# Autodesk Inventor assembly: 042-DXDE(F,D-166-3)
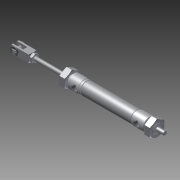
[picture p0: Inventor's stored thumbnail of the model, 180x180]
Saved by Autodesk Inventor 2012 (Build 160160000, 160)
## iProperties
Created: 2013-01-17
Part Number: 042-DXDE(F,D-166-3)
Catalog Web Link: www.cadenas.de
Description: Original Line Standard Air Cylinders-
Vendor: BIMBA
Document SubType Name: Assembly
Designer: William
Manufacturer: BIMBA
Category: PARTsolutions
Company: BIMBA
Title: 042-DXDE
Author: Cadenas PARTsolutions
PSOL_IDENT_0: {\\10.0.0.242\data_v9\23d-libs\bimba\bimba\bimba_imperial\bimba_full_line\original_line_cylinders\st
PSOL_IDENT_1: andard_air_cylinders\standard_air_cylinder_asmtab.prj},318 {VTYP=3D},{STYP=ASSTAB},{NB=042-DXDE(F,D-
PSOL_IDENT_2: 166-3)},{LINA=042-DXDE},{NN=Original Line Standard Air Cylinders},{DATE=06.09.2012 11:26:56},{GEOMDA
PSOL_IDENT_3: TE=06.09.2012},{VERSION=},{LINEID=50},{LINESUBID=-1},{WBVAR=STROKE,ACTING,MNT,DER,NR,BM,CO,OO,VO,M,E
PSOL_IDENT_4: E,EEL,K,Q,Y,G,T,B,H,SER,SR,NT,W,HL,STPT1,STPT2,STPT3,STPT4,MB,PB,PRC,TB,MN}  {NB=042-DXDE(F,D-166-3)
PSOL_IDENT_5: },{LINA=042-DXDE},{KT=DUMMY},{PN=042-DXDE},{PNC=042-DXDE(F,D-166-3)},{PNA=(D-166-3)},{DASH=-},{BORE1
PSOL_IDENT_6: =0.75000000},{BORE=3/4\" (04)},{BOREPN=04},{STROKE=2.000},{STROKEALG=[0.011:50/0.001]},{STROKE1=2.00
PSOL_IDENT_7: 0},{ACTING=D},{ACTINGALG= '' , 'Single Acting (SA)' , 'R' , 'Reverse Single Acting (SA)' , 'D' , 'Do
PSOL_IDENT_8: uble Acting (SA)' },{ACTINGPN=D},{MNT=X},{MNTALG= '' , 'Front Nose Mounting (SA)' , 'P' , 'Rear Pivo
PSOL_IDENT_9: t Mounting (SA)' , 'XP' , 'Double End or Pivot Mounting (SA)' , 'X' , 'Double End Mounting (SA)' , '
PSOL_IDENT_10: BF' , 'Front Block Mounting (SA)' , 'BR' , 'Rear Block Mounting for Vertical Positioning (SA)' , 'BF
PSOL_IDENT_11: T' , 'Front Block Trunnion Mounting (SA)' , 'BRT' , 'Rear Block Trunnion Mounting (SA)' },{TYPE=},{M
PSOL_IDENT_12: NTPN=X},{DER=DE},{DERALG= 'DE' , 'With Double End Rod' },{NR=},{NRALG= '' , 'N/A' },{NRPN=},{BM=},{B
PSOL_IDENT_13: MALG= '' , 'N/A' },{BMPN=},{CO=},{COALG= '' , 'N/A' },{OO=},{OOALG= '', 'N/A' },{OOPN=},{VO=Z},{VOAL
PSOL_IDENT_14: G= 'Z' , 'N/A' },{VOPN=},{OOVOPN=},{M=},{MALG= '', 'Without Magnet', 'M', 'With Magnet' },{EE=},{EEL
PSOL_IDENT_15: =0.000},{EEMAX=48.0000},{EEALG= '', 'Without Extra Extension', 'EE', 'With Extra Extension' },{EELAL
PSOL_IDENT_16: G=0},{EEPN=},{EEPN1=0.000},{K=},{KALG= '' , 'N/A' },{KPN=},{Q=},{QALG= '' , 'N/A' },{QPN=},{Y=},{YAL
PSOL_IDENT_17: G= '' , 'N/A' },{YPN=},{YCON=},{F=},{FALG= '', 'Non-Coated (Standard)', 'F', 'Molycoated' },{FPN=},{
PSOL_IDENT_18: G=},{GPN=},{GPN99=},{T=},{TALG= '' , 'Standard -20° to 200°F (-29° to 95°C)' , 'N' , 'Low Temperatur
PSOL_IDENT_19: e' , 'V' , 'High Temperature' },{NPN=},{VPN=},{B=},{BALG= '', 'W/out Bumpers' , 'B' , 'W/ Bumpers' }
PSOL_IDENT_20: ,{BPN=},{H=},{HALG= '', 'N/A' },{HPN=},{SER=},{SERALG= '' , 'Without Spring Return' , 'JS' , 'With S
PSOL_IDENT_21: pring Return' },{SR=},{SRALG= '' , 'Standard Stainless Steel' },{SRPN=},{SRCON=0},{NT=},{NTPN=},{W=}
PSOL_IDENT_22: ,{WALG= '' , 'Without Wiper' , 'W' , 'With Wiper' },{WPN=},{E=},{EALG= '' , 'Standard Seals/Lube' ,
PSOL_IDENT_23: 'E' , 'Non-Lube Seals/Lube' },{EPN=},{HL=},{HLALG= '' , 'Without Low Pressure Hydraulic' , 'HL' , 'W
PSOL_IDENT_24: ith Low Pressure Hydraulic' },{ST=},{STALG= '' , 'N/A' },{STPT1=},{STPT1ALG= '' , 'N/A' },{STPT2=},{
PSOL_IDENT_25: STPT2ALG= '' , 'N/A' },{STPT3=},{STPT3ALG= '' , 'N/A' },{STPT4=},{STPT4ALG= '' , 'N/A' },{STPN=},{MB
PSOL_IDENT_26: =},{MBALG= '' , 'Without Mounting Bracket' , 'F,D-129' , 'D-129 (front)'  , 'R,D-129' , 'D-129 (rear
PSOL_IDENT_27: )' , '2x,D-129' , 'D-129 (front & rear)'},{MBPN=},{MBPNALL=D-129},{MBPNALLREAR=D-129},{PB=},{PBALG=
PSOL_IDENT_28: '' , 'N/A' },{PBPN=},{PBPNALL=},{PRC=F,D-166-3},{PRCALG= '' , 'W/out Pivot Rod Clevis' , 'F,D-166-3'
PSOL_IDENT_29: , 'D-166-3 (front)' , 'R,D-166-3' , 'D-166-3 (rear)' , '2x,D-166-3' , 'D-166-3 (front & rear)' },{P
PSOL_IDENT_30: RCPN=(F,D-166-3)},{PRCPNALL=D-166-3},{TB=},{TBALG= '' , 'N/A' },{TBPN=},{TBPNALL=},{MN=},{MNALG= ''
PSOL_IDENT_31: , 'N/A' },{MNPN=},{MNCONF=},{MNCONR=},{TLEN=3.2570},{FRAC=9.0000},{RGCON=},{RGDACCON=R},{RHCON=DX},{
PSOL_IDENT_32: RHCON1=DX},{RHCONON=0},{RHACCON=},{FNUTCON=1},{RNUTCON=1},{FNUTPN=D-9},{RNUTPN=D-9},{FNUTTRANS=0.000
PSOL_IDENT_33: 0},{RNUTTRANS=0.0000},{VHOLECON=0},{A1=1.5940},{A1N=0.8750},{A1P=1.5940},{A1B=1.5940},{A4=0.2525},{A
PSOL_IDENT_34: 4N=0.3130},{A4P=0.2525},{A5=0.0300},{A1H=1.594},{A1NH=0.5310},{A1PH=1.5940},{A1BH=1.0940},{A1SH=1.21
PSOL_IDENT_35: 90},{A2H=0.2190},{A2NH=0.2190},{LENGTH=4.0000},{LENGTH1=4.0000},{LENGTH2=0.0000},{MUL=2.0000},{MUL11
PSOL_IDENT_36: =2.0000},{MUL22=5.38},{MUL33=5.3800},{MUL2=2.0000},{MUL211=2.0000},{MUL222=2.6900},{MUL233=2.6900},{
PSOL_IDENT_37: SSS=4.0000},{RGLEN=1.3715},{RHLEN=1.3715},{SSS1=3.0000},{A13=1.3120},{DIF=0.0000},{G5=0.6250},{ON=0}
PSOL_IDENT_38: ,{SSADD=0.0000},{BADD=0.0000},{MADD=0.0000},{NVADD=0.0000},{TRACKL=2.9670},{TRACKCON=D-74168},{TRIMC
PSOL_IDENT_39: ON=0},{TRIMCON1=0},{PINCON=},{FSPACE=0.6926},{SPACE=0.0643},{TEXT=0.1125},{S1=1.0000},{D1=0.8325},{D
PSOL_IDENT_40: 1N=0.8050},{D1B=0.8625},{D1P=0.8325},{FA=0.940},{RA=0.9400},{PPATH=standard_air_cylinder_asmtpl.prj}
PSOL_IDENT_41: ,{MATALGHTML=<b>Standard Original Line:</b><dl><dt>Rod:</dt><dd>- Stainless Steel</dd><dd>&nbsp;&nbs
PSOL_IDENT_42: p;(5/16  9/16 Bores)</dd><dd>- High Strength Carbon Steel</dd><dd>&nbsp;&nbsp;(3/4  3 Bore)</dd><d
PSOL_IDENT_43: d>- Stainless Steel</dd><dd>&nbsp;&nbsp;(X style DXP/DX/DXDE)</dd><dt>Bearings:</dt><dd>- Sintere
PSOL_IDENT_44: d Bronze</dd><dt>Body:</dt><dd>- 304 Stainless Steel</dd><dt>End Caps:</dt><dd>- Aluminum</dd><dt>Se
PSOL_IDENT_45: als:</dt><dd>- Buna N</dd></dl>},{ASSCFGPRA=04DXDE},{MBPNA=},{MNPNA=},{PRCPNA=(D-166-3)},{ASSOPTACC=
PSOL_IDENT_46: STPT4},{A=8.00},{HADD=0.0000},{WFL=0.25},{QADD=0.000},{QADD1=0.440},{TEST=2.0000},{MNTB=},{STDNUTF=1
PSOL_IDENT_47: },{STDNUTR=1}
CNS_NT: Standard Male Thread
CNS_NB: 042-DXDE(F,D-166-3)
CNS_NBSYN: $PNC.
CNS_LINA: 042-DXDE
CNS_PN: 042-DXDE
CNS_PNC: 042-DXDE(F,D-166-3)
CNS_PNA: (D-166-3)
CNS_DASH: -
CNS_BORE1: 0.75000000
CNS_BORE: 3/4" [04]
CNS_BOREPN: 04
CNS_STROKE: 2.000
CNS_STROKEALG: [0.011:50/0.001]
CNS_STROKE1: 2.000
CNS_ACTING: Double [D]
CNS_ACTINGALG: '' , 'Single Acting (SA)' , 'R' , 'Reverse Single Acting (SA)' , 'D' , 'Double Acting (SA)'
CNS_ACTINGPN: D
CNS_MNT: Double End [X]
CNS_MNTALG: '' , 'Front Nose Mounting (SA)' , 'P' , 'Rear Pivot Mounting (SA)' , 'XP' , 'Double End or Pivot Mounting (SA)' , 'X' , 'Double End Mounting (SA)' , 'BF' , 'Front Block Mounting (SA)' , 'BR' , 'Rear Block Mounting for Vertical Positioning (SA)' , 'BFT' , 'Front Block Trunnion Mounting (SA)' , 'BRT' , 'Rear Block Trunnion Mounting (SA)'
CNS_MNTPN: X
CNS_DER: Double End Rod [DE]
CNS_DERALG: 'DE' , 'With Double End Rod'
CNS_NR: N/A
CNS_NRALG: '' , 'N/A'
CNS_BM: N/A
CNS_BMALG: '' , 'N/A'
CNS_CO: N/A
CNS_COALG: '' , 'N/A'
CNS_OO: N/A
CNS_OOALG: '', 'N/A'
CNS_VO: N/A
CNS_VOALG: 'Z' , 'N/A'
CNS_M: Without Magnet Piston
CNS_MALG: '', 'Without Magnet', 'M', 'With Magnet'
CNS_EE: Standard Rod Extension
CNS_EEL: 0.000
CNS_EEMAX: 48.0000
CNS_EEALG: '', 'Without Extra Extension', 'EE', 'With Extra Extension'
CNS_EELALG: 0
CNS_EEPN1: 0.000
CNS_K: N/A
CNS_KALG: '' , 'N/A'
CNS_Q: N/A
CNS_QALG: '' , 'N/A'
CNS_Y: N/A
CNS_YALG: '' , 'N/A'
CNS_FALG: '', 'Non-Coated (Standard)', 'F', 'Molycoated'
CNS_G: Standard Grease Lube
CNS_T: Standard -20° to 200°F (-29° to 95°C)
CNS_TALG: '' , 'Standard -20° to 200°F (-29° to 95°C)' , 'N' , 'Low Temperature' , 'V' , 'High Temperature'
CNS_B: Without Bumpers
CNS_BALG: '', 'W/out Bumpers' , 'B' , 'W/ Bumpers'
CNS_H: N/A
CNS_HALG: '', 'N/A'
CNS_SER: Without Failsafe Spring Return
CNS_SERALG: '' , 'Without Spring Return' , 'JS' , 'With Spring Return'
CNS_SR: Standard Stainless Steel
CNS_SRALG: '' , 'Standard Stainless Steel'
CNS_SRCON: 0
CNS_W: Without Wiper
CNS_WALG: '' , 'Without Wiper' , 'W' , 'With Wiper'
CNS_EALG: '' , 'Standard Seals/Lube' , 'E' , 'Non-Lube Seals/Lube'
CNS_HL: Standard 250 PSI Air
CNS_HLALG: '' , 'Without Low Pressure Hydraulic' , 'HL' , 'With Low Pressure Hydraulic'
CNS_STALG: '' , 'N/A'
CNS_STPT1: N/A
CNS_STPT1ALG: '' , 'N/A'
CNS_STPT2: N/A
CNS_STPT2ALG: '' , 'N/A'
CNS_STPT3: N/A
CNS_STPT3ALG: '' , 'N/A'
CNS_STPT4: N/A
CNS_STPT4ALG: '' , 'N/A'
CNS_MB: Without Mounting Bracket
CNS_MBALG: '' , 'Without Mounting Bracket' , 'F,D-129' , 'D-129 (front)'  , 'R,D-129' , 'D-129 (rear)' , '2x,D-129' , 'D-129 (front & rear)'
CNS_MBPNALL: D-129
CNS_MBPNALLREAR: D-129
CNS_PB: N/A
CNS_PBALG: '' , 'N/A'
CNS_PRC: D-166-3 (front)
CNS_PRCALG: '' , 'W/out Pivot Rod Clevis' , 'F,D-166-3' , 'D-166-3 (front)' , 'R,D-166-3' , 'D-166-3 (rear)' , '2x,D-166-3' , 'D-166-3 (front & rear)'
CNS_PRCPN: (F,D-166-3)
CNS_PRCPNALL: D-166-3
CNS_TB: N/A
CNS_TBALG: '' , 'N/A'
CNS_MN: N/A
CNS_MNALG: '' , 'N/A'
CNS_TLEN: 3.2570
CNS_FRAC: 9.0000
CNS_RGDACCON: R
CNS_RHCON: DX
CNS_RHCON1: DX
CNS_RHCONON: 0
CNS_FNUTCON: 1
CNS_RNUTCON: 1
CNS_FNUTPN: D-9
CNS_RNUTPN: D-9
CNS_FNUTTRANS: 0.0000
CNS_RNUTTRANS: 0.0000
CNS_VHOLECON: 0
CNS_A1: 1.5940
CNS_A1N: 0.8750
CNS_A1P: 1.5940
CNS_A1B: 1.5940
CNS_A4: 0.2525
CNS_A4N: 0.3130
CNS_A4P: 0.2525
CNS_A5: 0.0300
CNS_A1H: 1.594
CNS_A1NH: 0.5310
CNS_A1PH: 1.5940
CNS_A1BH: 1.0940
CNS_A1SH: 1.2190
CNS_A2H: 0.2190
CNS_A2NH: 0.2190
CNS_LENGTH: 4.0000
CNS_LENGTH1: 4.0000
CNS_LENGTH2: 0.0000
CNS_MUL: 2.0000
CNS_MUL11: 2.0000
CNS_MUL22: 5.380
CNS_MUL33: 5.3800
CNS_MUL2: 2.0000
CNS_MUL211: 2.0000
CNS_MUL222: 2.6900
CNS_MUL233: 2.6900
CNS_SSS: 4.0000
CNS_RGLEN: 1.3715
CNS_RHLEN: 1.3715
CNS_SSS1: 3.0000
CNS_A13: 1.3120
CNS_DIF: 0.0000
CNS_G5: 0.6250
CNS_ON: 0
CNS_SSADD: 0.0000
CNS_BADD: 0.0000
CNS_MADD: 0.0000
CNS_NVADD: 0.0000
CNS_TRACKL: 2.9670
CNS_TRACKCON: D-74168
CNS_TRIMCON: 0
CNS_TRIMCON1: 0
CNS_FSPACE: 0.6926
CNS_SPACE: 0.0643
CNS_TEXT: 0.1125
CNS_S1: 1.0000
CNS_D1: 0.8325
CNS_D1N: 0.8050
CNS_D1B: 0.8625
CNS_D1P: 0.8325
CNS_FA: 0.940
CNS_RA: 0.9400
CNS_PPATH: standard_air_cylinder_asmtpl.prj
CNS_MATALGHTML: <b>Standard Original Line:</b><dl><dt>Rod:</dt><dd>- Stainless Steel</dd><dd>&nbsp;&nbsp;(5/16  9/16 Bores)</dd><dd>- High Strength Carbon Steel</dd><dd>&nbsp;&nbsp;(3/4  3 Bore)</dd><dd>- Stainless Steel</dd><dd>&nbsp;&nbsp;(X style DXP/DX/DXDE)</dd><dt>Bearings:</dt><dd>- Sintered Bronze</dd><dt>Body:</dt><dd>- 304 Stainless Steel</dd><dt>End Caps:</dt><dd>- Aluminum</dd><dt>Seals:</dt><dd>- Buna N</dd></dl>
CNS_ASSCFGPRA: 04DXDE
CNS_PRCPNA: (D-166-3)
CNS_ASSOPTACC: STPT4
CNS_A: 8.00
CNS_HADD: 0.0000
CNS_WFL: 0.250
CNS_QADD: 0.000
CNS_QADD1: 0.440
CNS_TEST: 2.0000
CNS_STDNUTF: 1
CNS_STDNUTR: 1
SUPPLIER: BIMBA
ARTICLENO: 042-DXDE(F,D-166-3)
BOMINFO: 042-DXDE
CREATOR: CADENAS GmbH
## Documents named in this file (10)
- C:\Users\William\Desktop\FRC CAD Files\Robot2013\Launcher\042-DXDE(F,D-166-3).iam
- C:\Users\William\Desktop\FRC CAD Files\Robot2013\Launcher\04R000_rod_guide.ipt
- C:\Users\William\Desktop\FRC CAD Files\Robot2013\Launcher\042-DXDE0_rod.ipt
- C:\Users\William\Desktop\FRC CAD Files\Robot2013\Launcher\D-166-3-dummy.ipt
- C:\Users\William\Desktop\FRC CAD Files\Robot2013\Launcher\D-14055.ipt
- C:\Users\William\Desktop\FRC CAD Files\Robot2013\Launcher\D-8381.ipt
- C:\Users\William\Desktop\FRC CAD Files\Robot2013\Launcher\D-5866.ipt
- C:\Users\William\Desktop\FRC CAD Files\Robot2013\Launcher\D-344.ipt
- C:\Users\William\Desktop\FRC CAD Files\Robot2013\Launcher\04R-3_2570.ipt
- C:\Users\William\Desktop\FRC CAD Files\Robot2013\Launcher\D-9.ipt
## Components (12 placed, 9 different names)
1. 04R000_rod_guide:1 — rod_guide_Z@1 <-> rod_cp_Z@2, to_tube_XY@1 <-> tube_front_XY@9, to_tube_Z@1 <-> tube_front_Z@9, to_tube_YZ@1 <-> tube_front_YZ@9, to_nut_XY@1 <-> NUT_XY@12, to_nut_Z@1 <-> NUT_Z@12, to_nut_YZ@1 <-> NUT_YZ@12
2. 042-DXDE0_rod:1 — rod_guide_Z@1 <-> rod_cp_Z@2
3. D-166-3-dummy:1 — dummy_XY@3 <-> dummy_XY@4, dummy_Z@3 <-> dummy_Z@4, dummy_YZ@3 <-> dummy_YZ@4
4. D-14055:1 — dummy_XY@3 <-> dummy_XY@4, dummy_Z@3 <-> dummy_Z@4, dummy_YZ@3 <-> dummy_YZ@4, rod_clevis_body_XY@4 <-> pin_XY@5, rod_clevis_body_Z@4 <-> pin_Z@5, piston_rod_clevis_XY@4 <-> NUT_XY@8, piston_rod_clevis_Z@4 <-> NUT_Z@8
5. D-8381:1 — rod_clevis_body_XY@4 <-> pin_XY@5, rod_clevis_body_Z@4 <-> pin_Z@5, rr1_XY@5 <-> RR_XY@6, rr1_Z@5 <-> RR_Z@6, rr2_XY@5 <-> RR_XY@7, rr2_Z@5 <-> RR_Z@7
6. D-5866:1 — rr1_XY@5 <-> RR_XY@6, rr1_Z@5 <-> RR_Z@6
7. D-5866:2 — rr2_XY@5 <-> RR_XY@7, rr2_Z@5 <-> RR_Z@7
8. D-344:1 — piston_rod_clevis_XY@4 <-> NUT_XY@8, piston_rod_clevis_Z@4 <-> NUT_Z@8
9. 04R-3_2570:1 — to_tube_XY@1 <-> tube_front_XY@9, to_tube_Z@1 <-> tube_front_Z@9, to_tube_YZ@1 <-> tube_front_YZ@9, tube_rear_XY@9 <-> to_tube_XY@10, tube_rear_Z@9 <-> to_tube_Z@10, tube_rear_YZ@9 <-> to_tube_YZ@10
10. 04R000_rod_guide:2 — tube_rear_XY@9 <-> to_tube_XY@10, tube_rear_Z@9 <-> to_tube_Z@10, tube_rear_YZ@9 <-> to_tube_YZ@10, to_nut_XY@10 <-> NUT_XY@11, to_nut_Z@10 <-> NUT_Z@11, to_nut_YZ@10 <-> NUT_YZ@11
11. D-9:1 — to_nut_XY@10 <-> NUT_XY@11, to_nut_Z@10 <-> NUT_Z@11, to_nut_YZ@10 <-> NUT_YZ@11
12. D-9:2 — to_nut_XY@1 <-> NUT_XY@12, to_nut_Z@1 <-> NUT_Z@12, to_nut_YZ@1 <-> NUT_YZ@12
## Relationships (24: Mate 16, Angle 5, Flush 3)
- rod_guide_Z@1 <-> rod_cp_Z@2 [Mate]: 04R000_rod_guide:1 ↔ 042-DXDE0_rod:1
- dummy_XY@3 <-> dummy_XY@4 [Mate]: D-166-3-dummy:1 ↔ D-14055:1
- dummy_Z@3 <-> dummy_Z@4 [Mate]: D-166-3-dummy:1 ↔ D-14055:1
- dummy_YZ@3 <-> dummy_YZ@4 [Angle] (0 deg): D-166-3-dummy:1 ↔ D-14055:1
- rod_clevis_body_XY@4 <-> pin_XY@5 [Mate]: D-14055:1 ↔ D-8381:1
- rod_clevis_body_Z@4 <-> pin_Z@5 [Mate]: D-14055:1 ↔ D-8381:1
- rr1_XY@5 <-> RR_XY@6 [Mate]: D-8381:1 ↔ D-5866:1
- rr1_Z@5 <-> RR_Z@6 [Mate]: D-8381:1 ↔ D-5866:1
- rr2_XY@5 <-> RR_XY@7 [Mate]: D-8381:1 ↔ D-5866:2
- rr2_Z@5 <-> RR_Z@7 [Mate]: D-8381:1 ↔ D-5866:2
- piston_rod_clevis_XY@4 <-> NUT_XY@8 [Mate]: D-14055:1 ↔ D-344:1
- piston_rod_clevis_Z@4 <-> NUT_Z@8 [Mate]: D-14055:1 ↔ D-344:1
- to_tube_XY@1 <-> tube_front_XY@9 [Flush]: 04R000_rod_guide:1 ↔ 04R-3_2570:1
- to_tube_Z@1 <-> tube_front_Z@9 [Mate]: 04R000_rod_guide:1 ↔ 04R-3_2570:1
- to_tube_YZ@1 <-> tube_front_YZ@9 [Angle] (0 deg): 04R000_rod_guide:1 ↔ 04R-3_2570:1
- tube_rear_XY@9 <-> to_tube_XY@10 [Mate]: 04R-3_2570:1 ↔ 04R000_rod_guide:2
- tube_rear_Z@9 <-> to_tube_Z@10 [Mate]: 04R-3_2570:1 ↔ 04R000_rod_guide:2
- tube_rear_YZ@9 <-> to_tube_YZ@10 [Angle] (0 deg): 04R-3_2570:1 ↔ 04R000_rod_guide:2
- to_nut_XY@10 <-> NUT_XY@11 [Flush]: 04R000_rod_guide:2 ↔ D-9:1
- to_nut_Z@10 <-> NUT_Z@11 [Mate]: 04R000_rod_guide:2 ↔ D-9:1
- to_nut_YZ@10 <-> NUT_YZ@11 [Angle] (0 deg): 04R000_rod_guide:2 ↔ D-9:1
- to_nut_XY@1 <-> NUT_XY@12 [Flush]: 04R000_rod_guide:1 ↔ D-9:2
- to_nut_Z@1 <-> NUT_Z@12 [Mate]: 04R000_rod_guide:1 ↔ D-9:2
- to_nut_YZ@1 <-> NUT_YZ@12 [Angle] (0 deg): 04R000_rod_guide:1 ↔ D-9:2
